# Autodesk Inventor assembly: BeltTightener_Assembly
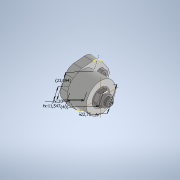
[picture p0: Inventor's stored thumbnail of the model, 180x180]
Saved by Autodesk Inventor 2021 (Build 250183000, 183)
## iProperties
Created: 2021-02-26
Part Number: BeltTightener_Assembly
Document SubType Name: Assembly
Designer: Viktor
Author: Viktor
## Documents named in this file (13)
- C:\Users\Viktor\Google Drive\Chalmers\Fortsatt arbete WR\Design files\Belt Tightener\BeltTightener_Assembly.iam
- C:\Users\Viktor\Google Drive\Chalmers\Fortsatt arbete WR\Design files\Belt Tightener\ISO 4762 - M6 x 12ISO.ipt
- C:\Users\Viktor\Google Drive\Chalmers\Fortsatt arbete WR\Design files\Belt Tightener\Bottom.ipt
- C:\Users\Viktor\Google Drive\Chalmers\Fortsatt arbete WR\Design files\Belt Tightener\DIN 125 - A 6,4.ipt
- C:\Users\Viktor\Google Drive\Chalmers\Fortsatt arbete WR\Design files\Belt Tightener\DIN 985 - M6.ipt
- C:\Users\Viktor\Google Drive\Chalmers\Fortsatt arbete WR\Design files\Belt Tightener\ISO 4762 - M5 x 8ISO.ipt
- C:\Users\Viktor\Google Drive\Chalmers\Fortsatt arbete WR\Design files\Belt Tightener\DIN 985 - M5.ipt
- C:\Users\Viktor\Google Drive\Chalmers\Fortsatt arbete WR\Design files\Belt Tightener\Roller.ipt
- C:\Users\Viktor\Google Drive\Chalmers\Fortsatt arbete WR\Design files\Belt Tightener\SS608-2RS.ipt
- C:\Users\Viktor\Google Drive\Chalmers\Fortsatt arbete WR\Design files\Belt Tightener\DIN 125 - A 8,4.ipt
- C:\Users\Viktor\Google Drive\Chalmers\Fortsatt arbete WR\Design files\Belt Tightener\DIN 985 - M8.ipt
- C:\Users\Viktor\Google Drive\Chalmers\Fortsatt arbete WR\Design files\Belt Tightener\DIN 933 - M8  x 35.ipt
- C:\Users\Viktor\Google Drive\Chalmers\Fortsatt arbete WR\Design files\Belt Tightener\Roller_Outer.ipt
## Components (16 placed, 12 different names)
1. ISO 4762 - M6 x 12ISO:1 — Rigid:1
2. Bottom:1 — Rotational:1, Rigid:2, Rigid:3, Rigid:4, Rotational:3, Rigid:12
3. DIN 125 - A 6,4:1 — Rigid:1, Rotational:1
4. DIN 985 - M6:1 — Rigid:2
5. ISO 4762 - M5 x 8ISO:1 — Rigid:3
6. DIN 985 - M5:1 — Rigid:4
7. Roller:1 — Rotational:2, Rigid:14
8. SS608-2RS:1 — Rigid:9, Rigid:10, Rotational:2
9. SS608-2RS:2 — Rigid:7, Rigid:8
10. DIN 125 - A 8,4:1 — Rigid:7, Rotational:3
11. DIN 125 - A 8,4:2 — Rigid:8, Rigid:11
12. DIN 125 - A 8,4:3 — Rigid:9, Rigid:11
13. DIN 125 - A 8,4:4 — Rigid:10, Rigid:13
14. DIN 933 - M8  x 35:1 — Rigid:12
15. DIN 985 - M8:1 — Rigid:13
16. Roller_Outer:1 — Rigid:14
## Relationships (15: WeldJoint 12, RevoluteJoint 3)
- Rigid:1 [WeldJoint]: ISO 4762 - M6 x 12ISO:1 ↔ DIN 125 - A 6,4:1
- Rotational:1 [RevoluteJoint] (-2 mm): Bottom:1 ↔ DIN 125 - A 6,4:1
- Rigid:2 [WeldJoint]: Bottom:1 ↔ DIN 985 - M6:1
- Rigid:3 [WeldJoint]: Bottom:1 ↔ ISO 4762 - M5 x 8ISO:1
- Rigid:4 [WeldJoint]: Bottom:1 ↔ DIN 985 - M5:1
- Rigid:7 [WeldJoint]: SS608-2RS:2 ↔ DIN 125 - A 8,4:1
- Rigid:8 [WeldJoint]: SS608-2RS:2 ↔ DIN 125 - A 8,4:2
- Rigid:9 [WeldJoint]: SS608-2RS:1 ↔ DIN 125 - A 8,4:3
- Rigid:10 [WeldJoint]: SS608-2RS:1 ↔ DIN 125 - A 8,4:4
- Rigid:11 [WeldJoint]: DIN 125 - A 8,4:2 ↔ DIN 125 - A 8,4:3
- Rotational:2 [RevoluteJoint] (-0.1 mm): Roller:1 ↔ SS608-2RS:1
- Rotational:3 [RevoluteJoint]: Bottom:1 ↔ DIN 125 - A 8,4:1
- Rigid:12 [WeldJoint]: Bottom:1 ↔ DIN 933 - M8  x 35:1
- Rigid:13 [WeldJoint]: DIN 125 - A 8,4:4 ↔ DIN 985 - M8:1
- Rigid:14 [WeldJoint]: Roller:1 ↔ Roller_Outer:1
